# Autodesk Inventor assembly: Pancake_Catch Assy_3 Lanes
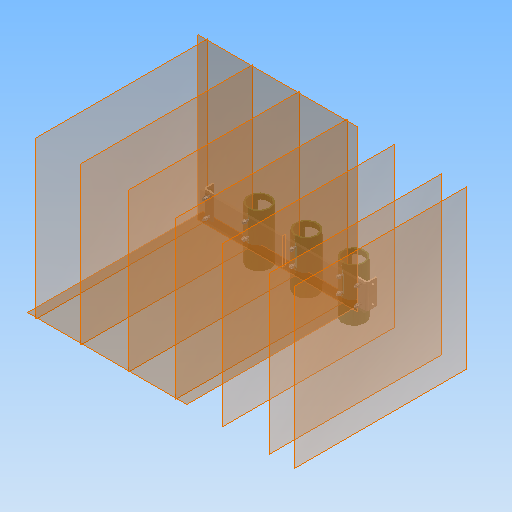
[picture p0: Inventor's stored thumbnail of the model, 512x512]
Saved by Autodesk Inventor 2018.1 (Build 221171000, 171)
## iProperties
Created: 2019-02-21
Part Number: Pancake_Catch Assy_3 Lanes
Document SubType Name: Assembly
Designer: James
Author: James
## Documents named in this file (7)
- C:\Users\admin\Desktop\Ball-Machine\Pancake Sort\Pancake - 3 Lanes\Pancake_Catch Assy_3 Lanes.iam
- C:\Users\admin\Desktop\Ball-Machine\Pancake Sort\Pancake_Catch Pipe.ipt
- C:\Users\admin\Desktop\Ball-Machine\Prototype CAD\Selection Sort - 40mm\Nyloc Nut - M4.ipt
- C:\Users\admin\Desktop\Ball-Machine\Prototype CAD\Selection Sort - 40mm\Socket Csk Screw - (A2) - M4 x  16.ipt
- C:\Users\admin\Desktop\Ball-Machine\Pancake Sort\Pancake_Angle Bracket.ipt
- C:\Users\admin\Desktop\Ball-Machine\Prototype CAD\Selection Sort - 40mm\Socket Cap Screw - Standard - (A2) - M4 x 16.ipt
- C:\Users\admin\Desktop\Ball-Machine\Pancake Sort\Pancake - 3 Lanes\Pancake_Catch Backboard_3 Lanes.ipt
## Components (26 placed, 6 different names)
1. Pancake_Catch Backboard_3 Lanes:1 — Flush:1, Flush:2, Flush:3, Tangent:1, Mate:1, Mate:2, Flush:4, Mate:5, Mate:6, Mate:9, Flush:6, Mate:10, Mate:11, Mate:12, Mate:13, Mate:14, Flush:7, Mate:19, Mate:20, Mate:27, Mate:28
2. Pancake_Angle Bracket:1 — Mate:9, Flush:6, Mate:10, Mate:11, Mate:23, Mate:24, Mate:25, Mate:26
3. Pancake_Angle Bracket:2 — Mate:12, Mate:13, Mate:14, Flush:7, Mate:15, Mate:16, Mate:17, Mate:18
4. Nyloc Nut - M4:11 — Mate:27, Mate:30
5. Socket Cap Screw - Standard - (A2) - M4 x 16:1 — Mate:23, Mate:25, Mate:29
6. Nyloc Nut - M4:12 — Mate:28, Mate:29
7. Socket Cap Screw - Standard - (A2) - M4 x 16:2 — Mate:24, Mate:26, Mate:30
8. Nyloc Nut - M4:13 — Mate:19, Mate:22
9. Socket Cap Screw - Standard - (A2) - M4 x 16:3 — Mate:17, Mate:18, Mate:21
10. Nyloc Nut - M4:14 — Mate:20, Mate:21
11. Socket Cap Screw - Standard - (A2) - M4 x 16:4 — Mate:15, Mate:16, Mate:22
12. Pancake_Catch Pipe:1 — Tangent:1, Mate:1, Mate:2, Mate:3, Mate:4, Angle:1
13. Nyloc Nut - M4:1 — Mate:5, Mate:8
14. Socket Csk Screw - (A2) - M4 x  16:1 — Mate:3, Flush:4, Flush:5, Mate:8
15. Nyloc Nut - M4:2 — Mate:6, Mate:7
16. Socket Csk Screw - (A2) - M4 x  16:2 — Mate:4, Flush:5, Mate:7
17. Pancake_Catch Pipe:2
18. Nyloc Nut - M4:3
19. Socket Csk Screw - (A2) - M4 x  16:3
20. Nyloc Nut - M4:4
21. Socket Csk Screw - (A2) - M4 x  16:4
22. Pancake_Catch Pipe:3
23. Nyloc Nut - M4:5
24. Socket Csk Screw - (A2) - M4 x  16:5
25. Nyloc Nut - M4:6
26. Socket Csk Screw - (A2) - M4 x  16:6
## Component patterns: (3 elements, first: Pancake_Catch Pipe:1 + Nyloc Nut - M4:1 + Socket Csk Screw - (A2) - M4 x  16:1 + Nyloc Nut - M4:2 + Socket Csk Screw - (A2) - M4 x  16:2)
## Relationships (39: Mate 30, Flush 7, Tangent 1, Angle 1)
- Flush:1: Pancake_Catch Backboard_3 Lanes:1
- Flush:2: Pancake_Catch Backboard_3 Lanes:1
- Flush:3: Pancake_Catch Backboard_3 Lanes:1
- Tangent:1: Pancake_Catch Backboard_3 Lanes:1 ↔ Pancake_Catch Pipe:1
- Mate:1: Pancake_Catch Backboard_3 Lanes:1 ↔ Pancake_Catch Pipe:1
- Mate:2: Pancake_Catch Backboard_3 Lanes:1 ↔ Pancake_Catch Pipe:1
- Mate:3: Pancake_Catch Pipe:1 ↔ Socket Csk Screw - (A2) - M4 x  16:1
- Mate:4: Pancake_Catch Pipe:1 ↔ Socket Csk Screw - (A2) - M4 x  16:2
- Flush:4 (-5 mm): Pancake_Catch Backboard_3 Lanes:1 ↔ Socket Csk Screw - (A2) - M4 x  16:1
- Flush:5: Socket Csk Screw - (A2) - M4 x  16:1 ↔ Socket Csk Screw - (A2) - M4 x  16:2
- Mate:5: Pancake_Catch Backboard_3 Lanes:1 ↔ Nyloc Nut - M4:1
- Mate:6: Pancake_Catch Backboard_3 Lanes:1 ↔ Nyloc Nut - M4:2
- Mate:7: Nyloc Nut - M4:2 ↔ Socket Csk Screw - (A2) - M4 x  16:2
- Mate:8: Nyloc Nut - M4:1 ↔ Socket Csk Screw - (A2) - M4 x  16:1
- Angle:1 (180 deg): Pancake_Catch Pipe:1
- Mate:9: Pancake_Catch Backboard_3 Lanes:1 ↔ Pancake_Angle Bracket:1
- Flush:6: Pancake_Catch Backboard_3 Lanes:1 ↔ Pancake_Angle Bracket:1
- Mate:10: Pancake_Catch Backboard_3 Lanes:1 ↔ Pancake_Angle Bracket:1
- Mate:11: Pancake_Catch Backboard_3 Lanes:1 ↔ Pancake_Angle Bracket:1
- Mate:12: Pancake_Catch Backboard_3 Lanes:1 ↔ Pancake_Angle Bracket:2
- Mate:13: Pancake_Catch Backboard_3 Lanes:1 ↔ Pancake_Angle Bracket:2
- Mate:14: Pancake_Catch Backboard_3 Lanes:1 ↔ Pancake_Angle Bracket:2
- Flush:7: Pancake_Catch Backboard_3 Lanes:1 ↔ Pancake_Angle Bracket:2
- Mate:15: Pancake_Angle Bracket:2 ↔ Socket Cap Screw - Standard - (A2) - M4 x 16:4
- Mate:16: Pancake_Angle Bracket:2 ↔ Socket Cap Screw - Standard - (A2) - M4 x 16:4
- Mate:17: Pancake_Angle Bracket:2 ↔ Socket Cap Screw - Standard - (A2) - M4 x 16:3
- Mate:18: Pancake_Angle Bracket:2 ↔ Socket Cap Screw - Standard - (A2) - M4 x 16:3
- Mate:19: Pancake_Catch Backboard_3 Lanes:1 ↔ Nyloc Nut - M4:13
- Mate:20: Pancake_Catch Backboard_3 Lanes:1 ↔ Nyloc Nut - M4:14
- Mate:21: Socket Cap Screw - Standard - (A2) - M4 x 16:3 ↔ Nyloc Nut - M4:14
- Mate:22: Nyloc Nut - M4:13 ↔ Socket Cap Screw - Standard - (A2) - M4 x 16:4
- Mate:23: Pancake_Angle Bracket:1 ↔ Socket Cap Screw - Standard - (A2) - M4 x 16:1
- Mate:24: Pancake_Angle Bracket:1 ↔ Socket Cap Screw - Standard - (A2) - M4 x 16:2
- Mate:25: Pancake_Angle Bracket:1 ↔ Socket Cap Screw - Standard - (A2) - M4 x 16:1
- Mate:26: Pancake_Angle Bracket:1 ↔ Socket Cap Screw - Standard - (A2) - M4 x 16:2
- Mate:27: Pancake_Catch Backboard_3 Lanes:1 ↔ Nyloc Nut - M4:11
- Mate:28: Pancake_Catch Backboard_3 Lanes:1 ↔ Nyloc Nut - M4:12
- Mate:29: Socket Cap Screw - Standard - (A2) - M4 x 16:1 ↔ Nyloc Nut - M4:12
- Mate:30: Nyloc Nut - M4:11 ↔ Socket Cap Screw - Standard - (A2) - M4 x 16:2
